# Autodesk Inventor assembly: A1-19027 Suction assembly
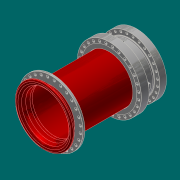
[picture p0: Inventor's stored thumbnail of the model, 180x180]
Saved by Autodesk Inventor 2017.3 (Build 213257000, 257)
## iProperties
Created: 2019-11-15
Part Number: A1-19027 Suction assembly
Document SubType Name: Assembly
Designer: GVD
Author: GVD
## Documents named in this file (3)
- N:\A1 - Projects\A1-19\A1-19027--Syncrude Aurora HT2 spools - SP-237\A1-19027 Suction assembly.iam
- N:\A1 - Projects\A1-19\A1-19027--Syncrude Aurora HT2 spools - SP-237\A1-19027-300-00 Spool SP-235-002-D-002-1.iam
- N:\A1 - Projects\A1-19\A1-19027--Syncrude Aurora HT2 spools - SP-237\A1-19027-500-00 Spool SP-235-002-D-002-1A.iam
## Components (2 placed, 2 different names)
1. A1-19027-300-00 Spool SP-235-002-D-002-1:1 [sub-assembly] — Insert:1, Angle:1
2. A1-19027-500-00 Spool SP-235-002-D-002-1A:1 [sub-assembly] — Insert:1, Angle:1
## Relationships (2: Insert 1, Angle 1)
- Insert:1: A1-19027-300-00 Spool SP-235-002-D-002-1:1 ↔ A1-19027-500-00 Spool SP-235-002-D-002-1A:1
- Angle:1 (0 deg): A1-19027-300-00 Spool SP-235-002-D-002-1:1 ↔ A1-19027-500-00 Spool SP-235-002-D-002-1A:1
